# Autodesk Inventor assembly: GFRP_T2_05
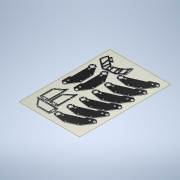
[picture p0: Inventor's stored thumbnail of the model, 180x180]
Saved by Autodesk Inventor 2022 (Build 260153000, 153)
## iProperties
Created: 2022-09-28
Part Number: GFRP_T2_05
Document SubType Name: Assembly
Designer: Masato
Author: Masato
## Documents named in this file (5)
- C:\Users\6343y\ドキュメント\Inventor\SUSTAINA-OP\Cam\GFRP_T2\OriginalMind_RD400\GFRP_T2_05.iam
- C:\Users\6343y\ドキュメント\Inventor\SUSTAINA-OP\Cam\DisposableBoard.ipt
- C:\Users\6343y\ドキュメント\Inventor\SUSTAINA-OP\UpperBody\Head\Head_neck_side_frame.ipt
- C:\Users\6343y\ドキュメント\Inventor\SUSTAINA-OP\LowerBody\Link\FrontLink_frame.ipt
- C:\Users\6343y\ドキュメント\Inventor\SUSTAINA-OP\UpperBody\Arm\UpperArm_side_frame.ipt
## Components (13 placed, 4 different names)
1. DisposableBoard:1 — フラッシュ:1, フラッシュ:2, フラッシュ:3, フラッシュ:4, 正接:4, 正接:5, フラッシュ:7, 正接:7, フラッシュ:8
2. Head_neck_side_frame:1 — メイト:11, 正接:7, 正接:8, 正接:9
3. UpperArm_side_frame:1 — メイト:13, メイト:15, メイト:17
4. UpperArm_side_frame:2 — メイト:14, メイト:16, メイト:17
5. UpperArm_side_frame:3 — メイト:12, フラッシュ:8, 正接:10, メイト:15, メイト:16
6. FrontLink_frame:3 — メイト:9, 正接:4, 正接:5, 正接:10
7. FrontLink_frame:12
8. FrontLink_frame:13
9. FrontLink_frame:14
10. FrontLink_frame:15
11. FrontLink_frame:16 — 正接:9
12. FrontLink_frame:17 — メイト:10, フラッシュ:7
13. FrontLink_frame:18 — 正接:8
## Component patterns: (6 elements, first: FrontLink_frame:3), (2 elements, first: FrontLink_frame:17)
## Relationships (21: Mate 9, Flush 6, Tangent 6)
- フラッシュ:1 [Flush]: DisposableBoard:1
- フラッシュ:2 [Flush]: DisposableBoard:1
- フラッシュ:3 [Flush]: DisposableBoard:1
- フラッシュ:4 [Flush]: DisposableBoard:1
- メイト:9 [Mate]: FrontLink_frame:3
- 正接:4 [Tangent] (2 mm): DisposableBoard:1 ↔ FrontLink_frame:3
- 正接:5 [Tangent] (2 mm): DisposableBoard:1 ↔ FrontLink_frame:3
- メイト:10 [Mate]: FrontLink_frame:17
- フラッシュ:7 [Flush] (2.1 mm): DisposableBoard:1 ↔ FrontLink_frame:17
- メイト:11 [Mate]: Head_neck_side_frame:1
- 正接:7 [Tangent] (2.1 mm): DisposableBoard:1 ↔ Head_neck_side_frame:1
- 正接:8 [Tangent] (2.1 mm): Head_neck_side_frame:1 ↔ FrontLink_frame:18
- 正接:9 [Tangent] (2.1 mm): Head_neck_side_frame:1 ↔ FrontLink_frame:16
- メイト:12 [Mate]: UpperArm_side_frame:3
- メイト:13 [Mate]: UpperArm_side_frame:1
- メイト:14 [Mate]: UpperArm_side_frame:2
- フラッシュ:8 [Flush] (2.1 mm): DisposableBoard:1 ↔ UpperArm_side_frame:3
- 正接:10 [Tangent] (2.1 mm): UpperArm_side_frame:3 ↔ FrontLink_frame:3
- メイト:15 [Mate] (2.1 mm): UpperArm_side_frame:1 ↔ UpperArm_side_frame:3
- メイト:16 [Mate] (2.1 mm): UpperArm_side_frame:2 ↔ UpperArm_side_frame:3
- メイト:17 [Mate] (2.1 mm): UpperArm_side_frame:1 ↔ UpperArm_side_frame:2
